# Autodesk Inventor assembly: POM_T5_01
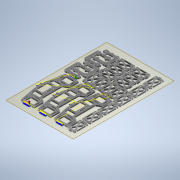
[picture p0: Inventor's stored thumbnail of the model, 180x180]
Saved by Autodesk Inventor 2022 (Build 260153000, 153)
## iProperties
Created: 2022-09-28
Part Number: POM_T5_01
Document SubType Name: Assembly
Designer: Masato
Author: Masato
## Documents named in this file (5)
- C:\Users\MasatoKubotera\Documents\Inventor\SUSTAINA-OP - CAM\Cam\POM_T5\OriginalMind_SR420\POM_T5_01.iam
- C:\Users\MasatoKubotera\Documents\Inventor\SUSTAINA-OP - CAM\Cam\DisposableBoard.ipt
- C:\Users\MasatoKubotera\Documents\Inventor\SUSTAINA-OP - CAM\UpperBody\Head\Head_camera_frame.ipt
- C:\Users\MasatoKubotera\Documents\Inventor\SUSTAINA-OP - CAM\UpperBody\Head\Head_neck_diagonal.ipt
- C:\Users\MasatoKubotera\Documents\Inventor\SUSTAINA-OP - CAM\UpperBody\Trunk\Trunk_chest_frame.iam
## Components (24 placed, 4 different names)
1. DisposableBoard:1 — フラッシュ:1, フラッシュ:2, フラッシュ:3, フラッシュ:4, フラッシュ:6, フラッシュ:9, フラッシュ:10
2. Head_camera_frame:1 — メイト:1, フラッシュ:6, メイト:3, 正接:1, フラッシュ:7, メイト:9
3. Head_camera_frame:2 — メイト:2, メイト:3, 正接:1, メイト:5
4. Head_camera_frame:3
5. Head_camera_frame:4
6. Trunk_chest_frame:1 [sub-assembly] — メイト:6, フラッシュ:9, フラッシュ:10, フラッシュ:8, メイト:9
7. Trunk_chest_frame:2 [sub-assembly]
8. Trunk_chest_frame:3 [sub-assembly]
9. Head_neck_diagonal:2 — フラッシュ:8, メイト:7, メイト:8
10. Head_neck_diagonal:3
11. Head_neck_diagonal:4
12. Head_neck_diagonal:5
13. Head_neck_diagonal:6
14. Head_neck_diagonal:7
15. Head_neck_diagonal:1 — メイト:4, フラッシュ:7, メイト:5, フラッシュ:11, メイト:11
16. Head_neck_diagonal:13
17. Head_neck_diagonal:14
18. Head_neck_diagonal:15 — メイト:8
19. Head_neck_diagonal:10 — メイト:10, フラッシュ:11, メイト:11
20. Head_neck_diagonal:16
21. Head_neck_diagonal:17
22. Head_neck_diagonal:18
23. Head_neck_diagonal:19
24. Head_neck_diagonal:20
## Component patterns: (2 elements, first: Head_camera_frame:1 + Head_camera_frame:2), (3 elements, first: Trunk_chest_frame:1), (6 elements, first: Head_neck_diagonal:2), (4 elements, first: Head_neck_diagonal:1), (6 elements, first: Head_neck_diagonal:10)
## Relationships (22: Mate 11, Flush 10, Tangent 1)
- フラッシュ:1 [Flush]: DisposableBoard:1
- フラッシュ:2 [Flush]: DisposableBoard:1
- フラッシュ:3 [Flush]: DisposableBoard:1
- フラッシュ:4 [Flush]: DisposableBoard:1
- メイト:1 [Mate]: Head_camera_frame:1
- フラッシュ:6 [Flush] (2 mm): DisposableBoard:1 ↔ Head_camera_frame:1
- メイト:2 [Mate]: Head_camera_frame:2
- メイト:3 [Mate] (2.1 mm): Head_camera_frame:1 ↔ Head_camera_frame:2
- 正接:1 [Tangent] (2.1 mm): Head_camera_frame:1 ↔ Head_camera_frame:2
- メイト:4 [Mate]: Head_neck_diagonal:1
- フラッシュ:7 [Flush]: Head_camera_frame:1 ↔ Head_neck_diagonal:1
- メイト:5 [Mate] (2.1 mm): Head_camera_frame:2 ↔ Head_neck_diagonal:1
- フラッシュ:8 [Flush]: Trunk_chest_frame:1 ↔ Head_neck_diagonal:2
- メイト:6 [Mate]: Trunk_chest_frame:1
- メイト:7 [Mate]: Head_neck_diagonal:2
- フラッシュ:9 [Flush] (-2 mm): DisposableBoard:1 ↔ Trunk_chest_frame:1
- フラッシュ:10 [Flush] (-2 mm): DisposableBoard:1 ↔ Trunk_chest_frame:1
- メイト:8 [Mate] (2.1 mm): Head_neck_diagonal:2 ↔ Head_neck_diagonal:15
- メイト:9 [Mate] (2.1 mm): Head_camera_frame:1 ↔ Trunk_chest_frame:1
- メイト:10 [Mate]: Head_neck_diagonal:10
- フラッシュ:11 [Flush]: Head_neck_diagonal:1 ↔ Head_neck_diagonal:10
- メイト:11 [Mate] (2.1 mm): Head_neck_diagonal:1 ↔ Head_neck_diagonal:10
